# Autodesk Inventor assembly: racked
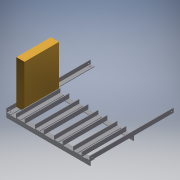
[picture p0: Inventor's stored thumbnail of the model, 180x180]
Saved by Autodesk Inventor 2017 (Build 210142000, 142)
## iProperties
Created: 2018-10-22
Part Number: racked
Document SubType Name: Assembly
Designer: ddeboer
Author: ddeboer
## Documents named in this file (3)
- C:\Users\ddeboer\Desktop\snap_holder\racked.iam
- C:\Users\ddeboer\Desktop\snap_holder\bottom.iam
- C:\Users\ddeboer\Desktop\snap_holder\snap.ipt
## Components (2 placed, 2 different names)
1. bottom:1 [sub-assembly] — Mate:1, Flush:1
2. snap:1 — Mate:1, Flush:1
## Relationships (2: Mate 1, Flush 1)
- Mate:1: bottom:1 ↔ snap:1
- Flush:1: bottom:1 ↔ snap:1
